# Autodesk Inventor assembly: HCMUTE-CDT23-FRAME_BTC_ASEMBLY
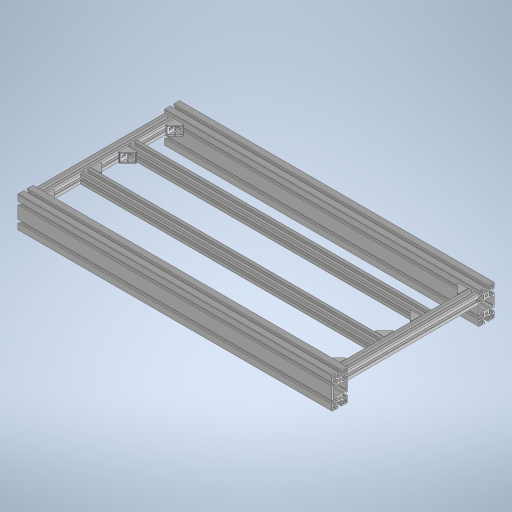
[picture p0: Inventor's stored thumbnail of the model, 512x512]
Saved by Autodesk Inventor 2023 (Build 270158000, 158)
## iProperties
Created: 2023-11-19
Part Number: HCMUTE-CDT23-FRAME_BTC_ASEMBLY
Document SubType Name: Assembly
Designer: havie
_SolveAssemblyDoc: Frame Generator Solve Assembly
_Version: 25.0.0
Author: havie
## Documents named in this file (4)
- C:\Users\havie\Desktop\DO_AN_CDT\1.1. PART\BANG_TAI_CAN\HCMUTE-CDT23-FRAME_BTC_ASEMBLY.iam
- C:\Users\havie\Desktop\DO_AN_CDT\1.1. PART\BANG_TAI_CAN\HCMUTE-CDT23-SKETCH_FRAME_BTC.ipt
- C:\Users\havie\Desktop\DO_AN_CDT\1.1. PART\BANG_TAI_CAN\HCMUTE-CDT23-FRAME_BTC_ASEMBLY\Frame\Frame 1700378415003.iam
- C:\Users\havie\Documents\Inventor\Content Center Files\R2023\en-US\301818\301818.ipt
## Components (10 placed, 3 different names)
1. HCMUTE-CDT23-SKETCH_FRAME_BTC:1
2. Frame 1700378415003:1 [sub-assembly] — Mate:1, Mate:2, Flush:1, Mate:3, Mate:4, Flush:2, Mate:5, Mate:6, Flush:3, Mate:7, Mate:8, Flush:4, Flush:5
3. 301818 302828.1:1 — Mate:3, Mate:4, Flush:2
4. 301818 302828.1:2 — Mate:1, Mate:2, Flush:1
5. 301818 302828.1:3 — Mate:7, Mate:8, Flush:4
6. 301818 302828.1:4 — Mate:5, Mate:6, Flush:3
7. 301818 302828.1:5
8. 301818 302828.1:6
9. 301818 302828.1:7
10. 301818 302828.1:8
## Relationships (13: Mate 8, Flush 5)
- Mate:1: Frame 1700378415003:1 ↔ 301818 302828.1:2
- Mate:2: Frame 1700378415003:1 ↔ 301818 302828.1:2
- Flush:1 (1 mm): Frame 1700378415003:1 ↔ 301818 302828.1:2
- Mate:3: Frame 1700378415003:1 ↔ 301818 302828.1:1
- Mate:4: Frame 1700378415003:1 ↔ 301818 302828.1:1
- Flush:2 (1 mm): Frame 1700378415003:1 ↔ 301818 302828.1:1
- Mate:5: Frame 1700378415003:1 ↔ 301818 302828.1:4
- Mate:6: Frame 1700378415003:1 ↔ 301818 302828.1:4
- Flush:3 (1 mm): Frame 1700378415003:1 ↔ 301818 302828.1:4
- Mate:7: Frame 1700378415003:1 ↔ 301818 302828.1:3
- Mate:8: Frame 1700378415003:1 ↔ 301818 302828.1:3
- Flush:4 (1 mm): Frame 1700378415003:1 ↔ 301818 302828.1:3
- Flush:5 (-300 mm): Frame 1700378415003:1
